# Autodesk Inventor assembly: 90_motor
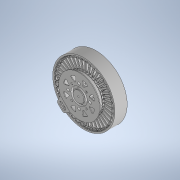
[picture p0: Inventor's stored thumbnail of the model, 180x180]
Saved by Autodesk Inventor 2020 (Build 240168000, 168)
## iProperties
Created: 2020-03-23
Part Number: 90_motor
Document SubType Name: Assembly
Designer: psrobotics
Author: psrobotics
## Documents named in this file (3)
- F:\projects-3\project dog gen3\hardware\belt_reducer\90_motor.iam
- F:\projects-3\project dog gen3\hardware\belt_reducer\90motor_base.ipt
- F:\projects-3\project dog gen3\hardware\belt_reducer\90motor_top.ipt
## Components (2 placed, 2 different names)
1. 90motor_base:1 — Insert:1
2. 90motor_top:1 — Insert:1
## Relationships (1: Insert 1)
- Insert:1 (-32.8 mm): 90motor_base:1 ↔ 90motor_top:1
